# Autodesk Inventor assembly: reducer_1
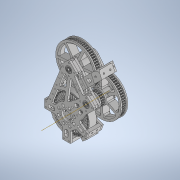
[picture p0: Inventor's stored thumbnail of the model, 180x180]
Saved by Autodesk Inventor 2020 (Build 240168000, 168)
## iProperties
Created: 2020-05-08
Part Number: reducer_1
Document SubType Name: Assembly
Designer: psrobotics
Author: psrobotics
## Documents named in this file (18)
- F:\projects-3\biped_gen1\hardware\reducer_1.iam
- F:\projects-3\biped_gen1\hardware\90_motor.iam
- F:\projects-3\biped_gen1\hardware\xl_20.ipt
- F:\projects-3\biped_gen1\hardware\xl_wheel_ass.iam
- F:\projects-3\biped_gen1\hardware\xl_60_out.ipt
- F:\projects-3\biped_gen1\hardware\motor_holder_1.ipt
- F:\projects-3\biped_gen1\hardware\bearing_8_16_5.ipt
- F:\projects-3\biped_gen1\hardware\pin_8_60.ipt
- F:\projects-3\biped_gen1\hardware\motor_holder_3.ipt
- F:\projects-3\biped_gen1\hardware\motor_holder_5.ipt
- F:\projects-3\biped_gen1\hardware\motor_holder_2.ipt
- F:\projects-3\biped_gen1\hardware\motor_holder_4.ipt
- F:\projects-3\biped_gen1\hardware\slide_holder_1.ipt
- F:\projects-3\biped_gen1\hardware\motor_holder_7.ipt
- F:\projects-3\biped_gen1\hardware\slide_holder_2.ipt
- F:\projects-3\biped_gen1\hardware\slide_holder_3.ipt
- F:\projects-3\biped_gen1\hardware\wheel_shift_1.ipt
- F:\projects-3\biped_gen1\hardware\motor_holder_6.ipt
## Components (24 placed, 17 different names)
1. 90_motor:1 [sub-assembly] — Insert:1, Insert:2, Insert:3, Insert:4
2. xl_20:1 — Insert:1, Insert:2, Flush:1, Tangent:1, Flush:3, Flush:4
3. xl_wheel_ass:1 [sub-assembly] — Flush:1, Tangent:1, Tangent:4, Flush:9, Insert:40
4. xl_60_out:1 — Insert:43
5. motor_holder_1:1 — Insert:3, Insert:4, Insert:5, Insert:17, Insert:18, Insert:22, Flush:5, Insert:24, Insert:25, Insert:26, Insert:27, Flush:6, Flush:10, Insert:41, Insert:42
6. bearing_8_16_5:1 — Insert:5, Insert:10
7. bearing_8_16_5:2 — Insert:15
8. pin_8_60:1 — Insert:10, Tangent:4
9. motor_holder_3:1 — Flush:3, Flush:4, Insert:28, Insert:29, Insert:32, Insert:33, Insert:38, Insert:39
10. motor_holder_5:1 — Insert:15, Insert:21, Insert:24, Insert:25, Flush:7, Flush:8, Insert:34, Insert:35, Insert:36, Insert:37
11. motor_holder_2:1 — Insert:17, Insert:18, Insert:19, Insert:20
12. motor_holder_4:1 — Insert:19, Insert:20, Insert:30, Insert:31
13. bearing_8_16_5:3 — Insert:21, Insert:43
14. bearing_8_16_5:4 — Insert:22, Insert:23
15. pin_8_60:2 — Insert:23
16. slide_holder_1:1 — Flush:5, Insert:26, Insert:27, Insert:28, Insert:29
17. motor_holder_7:1 — Insert:30, Insert:31
18. slide_holder_2:1 — Flush:7, Insert:32, Insert:33
19. slide_holder_3:1 — Flush:8, Insert:34, Insert:35
20. slide_holder_3:2 — Insert:36, Insert:37
21. bearing_8_16_5:5 — Insert:38
22. bearing_8_16_5:6 — Insert:39
23. wheel_shift_1:1 — Flush:9, Insert:40
24. motor_holder_6:1 — Flush:10, Insert:41, Insert:42
## Relationships (45: Insert 34, Flush 9, Tangent 2)
- Insert:1: 90_motor:1 ↔ xl_20:1
- Insert:2: 90_motor:1 ↔ xl_20:1
- Flush:1: xl_20:1 ↔ xl_wheel_ass:1
- Tangent:1 (2 mm): xl_20:1 ↔ xl_wheel_ass:1
- Insert:3: 90_motor:1 ↔ motor_holder_1:1
- Insert:4: 90_motor:1 ↔ motor_holder_1:1
- Insert:5: motor_holder_1:1 ↔ bearing_8_16_5:1
- Insert:10: bearing_8_16_5:1 ↔ pin_8_60:1
- Tangent:4 (-0.075 mm): xl_wheel_ass:1 ↔ pin_8_60:1
- Flush:3: xl_20:1 ↔ motor_holder_3:1
- Flush:4 (3 mm): xl_20:1 ↔ motor_holder_3:1
- Insert:15: bearing_8_16_5:2 ↔ motor_holder_5:1
- Insert:17: motor_holder_1:1 ↔ motor_holder_2:1
- Insert:18: motor_holder_1:1 ↔ motor_holder_2:1
- Insert:19: motor_holder_2:1 ↔ motor_holder_4:1
- Insert:20: motor_holder_2:1 ↔ motor_holder_4:1
- Insert:21: motor_holder_5:1 ↔ bearing_8_16_5:3
- Insert:22: motor_holder_1:1 ↔ bearing_8_16_5:4
- Insert:23: bearing_8_16_5:4 ↔ pin_8_60:2
- Flush:5: motor_holder_1:1 ↔ slide_holder_1:1
- Insert:24 (7 mm): motor_holder_1:1 ↔ motor_holder_5:1
- Insert:25 (7 mm): motor_holder_1:1 ↔ motor_holder_5:1
- Insert:26: motor_holder_1:1 ↔ slide_holder_1:1
- Insert:27: motor_holder_1:1 ↔ slide_holder_1:1
- Insert:28: motor_holder_3:1 ↔ slide_holder_1:1
- Insert:29: motor_holder_3:1 ↔ slide_holder_1:1
- Insert:30: motor_holder_4:1 ↔ motor_holder_7:1
- Insert:31: motor_holder_4:1 ↔ motor_holder_7:1
- Flush:6 (-40 mm): motor_holder_1:1
- Flush:7: motor_holder_5:1 ↔ slide_holder_2:1
- Insert:32: motor_holder_3:1 ↔ slide_holder_2:1
- Insert:33: motor_holder_3:1 ↔ slide_holder_2:1
- Flush:8: motor_holder_5:1 ↔ slide_holder_3:1
- Insert:34: motor_holder_5:1 ↔ slide_holder_3:1
- Insert:35: motor_holder_5:1 ↔ slide_holder_3:1
- Insert:36: motor_holder_5:1 ↔ slide_holder_3:2
- Insert:37: motor_holder_5:1 ↔ slide_holder_3:2
- Insert:38: motor_holder_3:1 ↔ bearing_8_16_5:5
- Insert:39: motor_holder_3:1 ↔ bearing_8_16_5:6
- Flush:9: xl_wheel_ass:1 ↔ wheel_shift_1:1
- Insert:40: xl_wheel_ass:1 ↔ wheel_shift_1:1
- Flush:10: motor_holder_1:1 ↔ motor_holder_6:1
- Insert:41: motor_holder_1:1 ↔ motor_holder_6:1
- Insert:42: motor_holder_1:1 ↔ motor_holder_6:1
- Insert:43 (0.7 mm): xl_60_out:1 ↔ bearing_8_16_5:3
